# Autodesk Inventor assembly: 5A.00.01.01-IB-VTP-Master-Assy
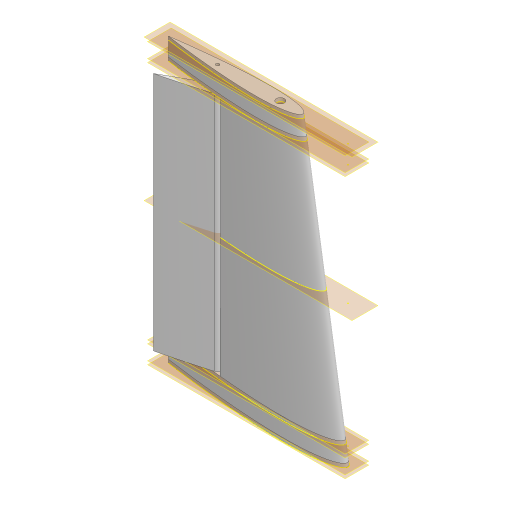
[picture p0: Inventor's stored thumbnail of the model, 512x512]
Saved by Autodesk Inventor 2024.3 (Build 283343000, 343)
## iProperties
Created: 2024-11-03
Part Number: 5A.00.01.01-IB-VTP-Master-Assy
Document SubType Name: Assembly
Designer: inigo
Author: inigo
## Documents named in this file (3)
- C:\Users\inigo\OneDrive - University of Bristol\General - grp-Company A - AVDASI2 2024-25\CAD Files\VTP\5A.00.01.01-IB-VTP-Master-Assy.iam
- C:\Users\inigo\OneDrive - University of Bristol\General - grp-Company A - AVDASI2 2024-25\CAD Files\VTP\5P.00.01.01-IB-VTP-Body.ipt
- C:\Users\inigo\OneDrive - University of Bristol\General - grp-Company A - AVDASI2 2024-25\CAD Files\VTP\5P.00.01.01-IB-VTP-Rudder.ipt
## Components (2 placed, 2 different names)
1. 5P.00.01.01-IB-VTP-Body:1 — Mate:1, Mate:2, Flush:1, Flush:2
2. 5P.00.01.01-IB-VTP-Rudder:1 — Mate:1, Mate:2, Mate:3
## Relationships (5: Mate 3, Flush 2)
- Mate:1: 5P.00.01.01-IB-VTP-Body:1 ↔ 5P.00.01.01-IB-VTP-Rudder:1
- Mate:2: 5P.00.01.01-IB-VTP-Body:1 ↔ 5P.00.01.01-IB-VTP-Rudder:1
- Mate:3: 5P.00.01.01-IB-VTP-Rudder:1
- Flush:1: 5P.00.01.01-IB-VTP-Body:1
- Flush:2: 5P.00.01.01-IB-VTP-Body:1
